# Autodesk Inventor assembly: CAR_021_BracePattern
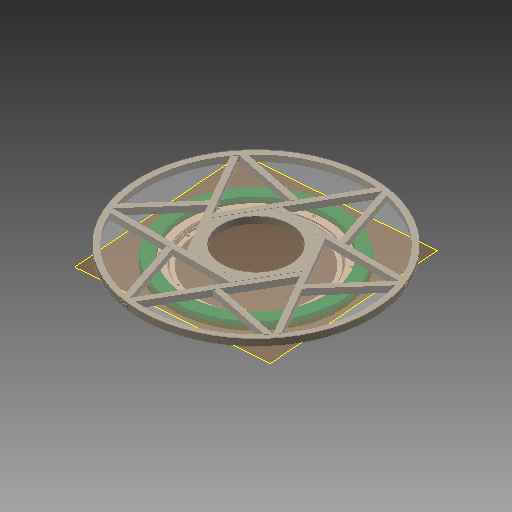
[picture p0: Inventor's stored thumbnail of the model, 512x512]
Saved by Autodesk Inventor 2018.3 (Build 223284000, 284)
## iProperties
Created: 2020-01-31
Part Number: CAR_021_BracePattern
Document SubType Name: Assembly
Designer: dillmcke
Mass: 2195.94 g
Surface Area: 13399.9 cm^2
Volume: 2315.72 cm^3
Density: 0.948274 g/cm^3
Author: dillmcke
## Documents named in this file (10)
- C:\Users\22turnmaxw\Documents\GrabCAD\Infinite Recharge 2020\Build season\CAR_021_BracePattern.iam
- C:\Users\22turnmaxw\Documents\GrabCAD\Infinite Recharge 2020\Brainstorming\CarouselSkin2\CarouselSkinCenter2.ipt
- C:\Users\22turnmaxw\Documents\GrabCAD\Infinite Recharge 2020\Brainstorming\CarouselSkin2\CarouselSkin2OuterRim.ipt
- C:\Users\22turnmaxw\Documents\GrabCAD\Infinite Recharge 2020\Brainstorming\CarouselSkin2\CarouselSkin2_HexLeg.ipt
- C:\Users\22turnmaxw\Documents\GrabCAD\Infinite Recharge 2020\Build season\CAR_001_McMaster Carr 18635A520_ROUND TURNTABLE.ipt
- C:\Users\22turnmaxw\Documents\GrabCAD\Infinite Recharge 2020\Brainstorming\CarouselSkin2\CarouselGearLowFi.ipt
- C:\Users\22turnmaxw\Documents\GrabCAD\Infinite Recharge 2020\Brainstorming\CarouselSkin2\CarouselSkin2_ShortStrut.ipt
- C:\Users\22turnmaxw\Documents\GrabCAD\Infinite Recharge 2020\Brainstorming\CarouselSkin2\CarouselSkin2_OuterRimSigmentMid.ipt
- C:\Users\22turnmaxw\Documents\GrabCAD\Infinite Recharge 2020\Brainstorming\CarouselSkin2\CarouselSkin2_LexanCircle.ipt
- C:\Users\22turnmaxw\Documents\GrabCAD\Infinite Recharge 2020\Brainstorming\CarouselSkin2\CarouselSkin2_LexanCircle_MIR.ipt
## Components (19 placed, 9 different names)
1. CarouselSkinCenter2:1 — Flush:1, Mate:1, Flush:2, Mate:3, Mate:9
2. CarouselSkin2OuterRim:1 — Flush:1, Mate:1, Flush:4, Flush:5, Flush:6, Symmetry:1, Mate:8
3. CAR_001_McMaster Carr 18635A520_ROUND TURNTABLE:1 — Mate:3, Mate:5, Flush:7
4. CarouselGearLowFi:1 — Mate:5, Mate:7, Flush:7
5. CarouselSkin2_OuterRimSigmentMid:1 — Flush:4, Flush:5
6. CarouselSkin2_LexanCircle:1 — Flush:6, Symmetry:1
7. CarouselSkin2_LexanCircle_MIR:1 — Mate:7, Mate:8, Mate:9
8. CarouselSkin2_HexLeg:1 — Flush:2
9. CarouselSkin2_HexLeg:2
10. CarouselSkin2_HexLeg:3
11. CarouselSkin2_HexLeg:4
12. CarouselSkin2_HexLeg:5
13. CarouselSkin2_HexLeg:6 — Flush:3
14. CarouselSkin2_ShortStrut:1 — Flush:3
15. CarouselSkin2_ShortStrut:2
16. CarouselSkin2_ShortStrut:3
17. CarouselSkin2_ShortStrut:4
18. CarouselSkin2_ShortStrut:5
19. CarouselSkin2_ShortStrut:6
## Component patterns: (6 elements, first: CarouselSkin2_HexLeg:1), (6 elements, first: CarouselSkin2_ShortStrut:1)
## Relationships (14: Flush 7, Mate 6, Symmetry 1)
- Flush:1: CarouselSkinCenter2:1 ↔ CarouselSkin2OuterRim:1
- Mate:1: CarouselSkinCenter2:1 ↔ CarouselSkin2OuterRim:1
- Flush:2: CarouselSkinCenter2:1 ↔ CarouselSkin2_HexLeg:1
- Mate:3: CarouselSkinCenter2:1 ↔ CAR_001_McMaster Carr 18635A520_ROUND TURNTABLE:1
- Mate:5: CAR_001_McMaster Carr 18635A520_ROUND TURNTABLE:1 ↔ CarouselGearLowFi:1
- Flush:3: CarouselSkin2_HexLeg:6 ↔ CarouselSkin2_ShortStrut:1
- Flush:4: CarouselSkin2OuterRim:1 ↔ CarouselSkin2_OuterRimSigmentMid:1
- Flush:5: CarouselSkin2OuterRim:1 ↔ CarouselSkin2_OuterRimSigmentMid:1
- Flush:6: CarouselSkin2OuterRim:1 ↔ CarouselSkin2_LexanCircle:1
- Symmetry:1: CarouselSkin2OuterRim:1 ↔ CarouselSkin2_LexanCircle:1
- Mate:7 (3.175 mm): CarouselGearLowFi:1 ↔ CarouselSkin2_LexanCircle_MIR:1
- Mate:8: CarouselSkin2OuterRim:1 ↔ CarouselSkin2_LexanCircle_MIR:1
- Mate:9: CarouselSkinCenter2:1 ↔ CarouselSkin2_LexanCircle_MIR:1
- Flush:7 (12.7 mm): CAR_001_McMaster Carr 18635A520_ROUND TURNTABLE:1 ↔ CarouselGearLowFi:1
